# Autodesk Inventor assembly: s-assy-gripper
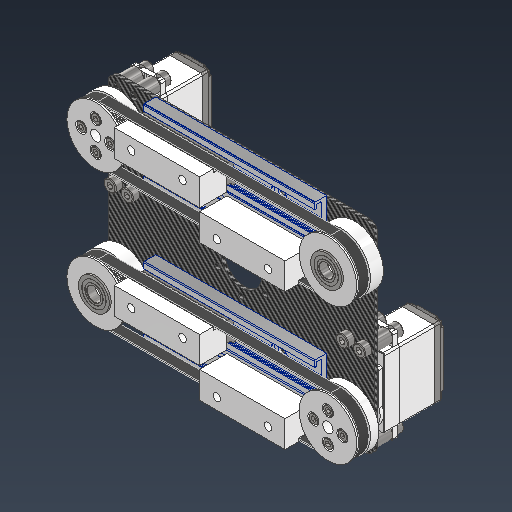
[picture p0: Inventor's stored thumbnail of the model, 512x512]
Saved by Autodesk Inventor 2021 (Build 250183000, 183)
## iProperties
Created: 2021-08-06
Part Number: s-assy-gripper
Document SubType Name: Assembly
Designer: yuta0
Mass: 234.241 g
Surface Area: 929.587 cm^2
Volume: 118.773 cm^3
Density: 1.97217 g/cm^3
Author: yuta0
## Documents named in this file (14)
- C:\Users\yuta0\Documents\GitHub\catchrobo_hardware\catchrobo_robot\s-assy-gripper.iam
- C:\Users\yuta0\Documents\GitHub\catchrobo_hardware\catchrobo_robot\carbon_plate14.ipt
- C:\Users\yuta0\Downloads\新しいフォルダー\MG_996R.iam
- C:\Users\yuta0\Downloads\新しいフォルダー\mrs20-100.ipt
- C:\Users\yuta0\Downloads\新しいフォルダー\mr-20cs_1.iam
- C:\Users\yuta0\Documents\GitHub\catchrobo_hardware\catchrobo_robot\base35.ipt
- C:\Users\yuta0\Documents\GitHub\catchrobo_hardware\catchrobo_robot\belt4.ipt
- C:\Users\yuta0\Documents\GitHub\catchrobo_hardware\catchrobo_robot\base36.ipt
- C:\Users\yuta0\Documents\GitHub\catchrobo_hardware\catchrobo_robot\FL688ZZ.ipt
- C:\Users\yuta0\Documents\GitHub\catchrobo_hardware\catchrobo_robot\ARF-410E.ipt
- C:\Users\yuta0\Documents\GitHub\catchrobo_hardware\catchrobo_robot\CB4-6.ipt
- C:\Users\yuta0\Documents\GitHub\catchrobo_hardware\catchrobo_robot\CC-0814-05.ipt
- C:\Users\yuta0\Desktop\lab\gripper_adapter-20201120T022136Z-001\gripper_adapter\CB3-12.ipt
- C:\Users\yuta0\Documents\GitHub\catchrobo_hardware\catchrobo_robot\base37.ipt
## Components (55 placed, 13 different names)
1. carbon_plate14:1 — メイト:1, メイト:2, メイト:3, メイト:11, メイト:12, メイト:16, メイト:27, メイト:33, メイト:36, メイト:37
2. FL688ZZ:2 — メイト:29, メイト:30, メイト:39
3. FL688ZZ:1 — メイト:26, メイト:27, メイト:28, メイト:38
4. base36:1 — メイト:24, メイト:25, メイト:26, メイト:28, メイト:29, メイト:30
5. belt4:1 — メイト:20, メイト:21, メイト:24, メイト:25
6. mr-20cs_1:2 [sub-assembly] — フラッシュ:2, メイト:31, フラッシュ:3, メイト:48, メイト:49, メイト:50
7. mr-20cs_1:1 [sub-assembly] — メイト:7, メイト:8, フラッシュ:1, フラッシュ:2, メイト:45, メイト:46, メイト:47
8. base35:1 — メイト:17, メイト:18, メイト:19, メイト:20, メイト:21, メイト:43, メイト:44
9. MG_996R:1 [sub-assembly] — メイト:11, メイト:12, メイト:16, メイト:17, メイト:18, メイト:19, メイト:32, メイト:34, メイト:35
10. CC-0814-05:1 — メイト:38, メイト:39
11. base37:1 — メイト:45, メイト:46, メイト:47
12. base37:2 — メイト:48, メイト:49, メイト:50
13. FL688ZZ:3
14. FL688ZZ:4
15. base36:2
16. belt4:2
17. mr-20cs_1:3 [sub-assembly]
18. mr-20cs_1:4 [sub-assembly]
19. base35:2
20. MG_996R:2 [sub-assembly]
21. CC-0814-05:2
22. base37:3
23. base37:4
24. mrs20-100:1 — メイト:1, メイト:2, メイト:3, メイト:7, メイト:8, フラッシュ:1
25. mrs20-100:2 — メイト:31, フラッシュ:3
26. ARF-410E:1 — メイト:32, メイト:33
27. CB4-6:1 — メイト:34, メイト:35
28. ARF-410E:2
29. CB4-6:2
30. ARF-410E:3
31. CB4-6:3
32. ARF-410E:4
33. CB4-6:4
34. CB4-6:5 — メイト:36, メイト:37
35. CB4-6:6
36. CB3-12:1 — メイト:43, メイト:44
37. CB3-12:2
38. CB3-12:3
39. CB3-12:4
40. mrs20-100:3
41. mrs20-100:4
42. ARF-410E:5
43. CB4-6:7
44. ARF-410E:6
45. CB4-6:8
46. ARF-410E:7
47. CB4-6:9
48. ARF-410E:8
49. CB4-6:10
50. CB4-6:11
51. CB4-6:12
52. CB3-12:5
53. CB3-12:6
54. CB3-12:7
55. CB3-12:8
## Component patterns: (2 elements, first: FL688ZZ:2 + FL688ZZ:1 + base36:1 + belt4:1 + mr-20cs_1:2 + mr-20cs_1:1 + base35:1 + MG_996R:1 + CC-0814-05:1 + base37:1 + base37:2), (2 elements, first: mrs20-100:1), (4 elements, first: ARF-410E:1 + CB4-6:1), (2 elements, first: CB4-6:5), (4 elements, first: CB3-12:1), コンポーネント パターン 4:2 (2 elements), コンポーネント パターン 5:2 (4 elements), コンポーネント パターン 7:2 (2 elements), コンポーネント パターン 8:2 (4 elements)
## Relationships (40: Mate 37, Flush 3)
- メイト:1 [Mate]: carbon_plate14:1 ↔ mrs20-100:1
- メイト:2 [Mate]: carbon_plate14:1 ↔ mrs20-100:1
- メイト:3 [Mate]: carbon_plate14:1 ↔ mrs20-100:1
- メイト:7 [Mate] (0.1 mm): mr-20cs_1:1 ↔ mrs20-100:1
- メイト:8 [Mate] (0.15 mm): mr-20cs_1:1 ↔ mrs20-100:1
- フラッシュ:1 [Flush]: mr-20cs_1:1 ↔ mrs20-100:1
- メイト:11 [Mate]: carbon_plate14:1 ↔ MG_996R:1
- メイト:12 [Mate]: carbon_plate14:1 ↔ MG_996R:1
- メイト:16 [Mate] (10 mm): carbon_plate14:1 ↔ MG_996R:1
- メイト:17 [Mate]: base35:1 ↔ MG_996R:1
- メイト:18 [Mate]: base35:1 ↔ MG_996R:1
- メイト:19 [Mate]: base35:1 ↔ MG_996R:1
- メイト:20 [Mate]: belt4:1 ↔ base35:1
- メイト:21 [Mate] (0.5 mm): belt4:1 ↔ base35:1
- メイト:24 [Mate]: base36:1 ↔ belt4:1
- メイト:25 [Mate] (0.5 mm): base36:1 ↔ belt4:1
- メイト:26 [Mate]: FL688ZZ:1 ↔ base36:1
- メイト:27 [Mate]: carbon_plate14:1 ↔ FL688ZZ:1
- メイト:28 [Mate]: FL688ZZ:1 ↔ base36:1
- メイト:29 [Mate]: FL688ZZ:2 ↔ base36:1
- メイト:30 [Mate]: FL688ZZ:2 ↔ base36:1
- フラッシュ:2 [Flush]: mr-20cs_1:2 ↔ mr-20cs_1:1
- メイト:31 [Mate] (0.1 mm): mr-20cs_1:2 ↔ mrs20-100:2
- フラッシュ:3 [Flush]: mr-20cs_1:2 ↔ mrs20-100:2
- メイト:32 [Mate]: MG_996R:1 ↔ ARF-410E:1
- メイト:33 [Mate]: carbon_plate14:1 ↔ ARF-410E:1
- メイト:34 [Mate]: MG_996R:1 ↔ CB4-6:1
- メイト:35 [Mate]: MG_996R:1 ↔ CB4-6:1
- メイト:36 [Mate]: carbon_plate14:1 ↔ CB4-6:5
- メイト:37 [Mate]: carbon_plate14:1 ↔ CB4-6:5
- メイト:38 [Mate]: FL688ZZ:1 ↔ CC-0814-05:1
- メイト:39 [Mate]: FL688ZZ:2 ↔ CC-0814-05:1
- メイト:43 [Mate]: base35:1 ↔ CB3-12:1
- メイト:44 [Mate]: base35:1 ↔ CB3-12:1
- メイト:45 [Mate]: mr-20cs_1:1 ↔ base37:1
- メイト:46 [Mate]: mr-20cs_1:1 ↔ base37:1
- メイト:47 [Mate]: mr-20cs_1:1 ↔ base37:1
- メイト:48 [Mate]: mr-20cs_1:2 ↔ base37:2
- メイト:49 [Mate]: mr-20cs_1:2 ↔ base37:2
- メイト:50 [Mate]: mr-20cs_1:2 ↔ base37:2
